# Autodesk Inventor assembly: robotface
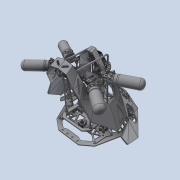
[picture p0: Inventor's stored thumbnail of the model, 180x180]
Saved by Autodesk Inventor 2020 (Build 240168000, 168)
## iProperties
Created: 2021-06-30
Part Number: robotface
Document SubType Name: Assembly
Designer: valer
Author: valer
## Documents named in this file (47)
- C:\Users\Val\Desktop\drummingrobot\design\robotface\robotface.iam
- C:\Users\Val\Desktop\drummingrobot\design\robotface\robotface-final.ipt
- C:\Users\Val\Desktop\drummingrobot\src\parts\external\HingedThreadedStandoffPart2.ipt
- C:\Users\Val\Desktop\drummingrobot\src\parts\external\HingedThreadedStandoffPart1.ipt
- C:\Users\Val\Desktop\drummingrobot\design\robotface\TongueMount.ipt
- C:\Users\Val\Desktop\drummingrobot\design\robotface\HeadMount.ipt
- C:\Users\Val\Desktop\drummingrobot\design\robotface\LinearBearing-1612-0612-0035.ipt
- C:\Users\Val\Desktop\drummingrobot\design\robotface\ClampingHub1301-0016-0012.ipt
- C:\Users\Val\Desktop\drummingrobot\design\robotface\UJoint6D\UJoint6D-Body-4003-1006-1006.ipt
- C:\Users\Val\Desktop\drummingrobot\design\robotface\UJoint6D\UJoint6D-CenterDrive-4003-1006-1006.ipt
- C:\Users\Val\Desktop\drummingrobot\design\robotface\UJoint6D\UJoint6D-Screw.ipt
- C:\Users\Val\Desktop\drummingrobot\design\robotface\SetScrewLiteHub-1308-0016-0006.ipt
- C:\Users\Val\Desktop\drummingrobot\design\robotface\ShaftD6-Short-2101-0006-0020.ipt
- C:\Users\Val\Desktop\drummingrobot\design\robotface\SetScrewHub-1300-0016-1006.ipt
- C:\Users\Val\Desktop\drummingrobot\design\robotface\ShaftD6Female-632Female.ipt
- C:\Users\Val\Desktop\drummingrobot\design\robotface\ShaftD6-2101-0006-0160.ipt
- C:\Users\Val\Desktop\drummingrobot\design\robotface\HeadTongueMount.ipt
- C:\Users\Val\Desktop\drummingrobot\design\robotface\Rod4mm.ipt
- C:\Users\Val\Desktop\drummingrobot\design\robotface\NoseBentBar.ipt
- C:\Users\Val\Desktop\drummingrobot\design\robotface\HeadTopConnector.ipt
- C:\Users\Val\Desktop\drummingrobot\design\robotface\UJointSq-4005-0016-0001\4005-0016-0001 Outer Shell.ipt
- C:\Users\Val\Desktop\drummingrobot\design\robotface\RodEndFixed-2434K495_CORROSION-RESISTANT FULLY THREADED ROD END BOLT.ipt
- C:\Users\Val\Desktop\drummingrobot\design\robotface\StandoffM4-1501-0006-0420.ipt
- C:\Users\Val\Desktop\drummingrobot\design\robotface\StandoffM4-1501-0006-0340.ipt
- C:\Users\Val\Desktop\drummingrobot\src\parts\external\Arducam.ipt
- C:\Users\Val\Desktop\drummingrobot\src\parts\external\ArducamHat.ipt
- C:\Users\Val\Desktop\drummingrobot\design\robotface\HeadEyeMount.ipt
- C:\Users\Val\Desktop\drummingrobot\design\robotface\M3-Standoff-30mm.ipt
- C:\Users\Val\Desktop\drummingrobot\design\robotface\M5-Standoff-32mm.ipt
- C:\Users\Val\Desktop\drummingrobot\src\parts\external\ArducamMirror.ipt
- C:\Users\Val\Desktop\drummingrobot\design\robotface\M1-Standoff-20mm.ipt
- C:\Users\Val\Desktop\drummingrobot\design\robotface\NoseInsideConnector.ipt
- C:\Users\Val\Desktop\drummingrobot\design\robotface\Part2^3mm U-Joint.ipt
- C:\Users\Val\Desktop\drummingrobot\design\robotface\Part1^3mm U-Joint.ipt
- C:\Users\Val\Desktop\drummingrobot\design\robotface\NoseCover.ipt
- C:\Users\Val\Desktop\drummingrobot\design\robotface\NoseCoverSmall.ipt
- C:\Users\Val\Desktop\drummingrobot\design\robotface\IRLed-FY-4006.ipt
- C:\Users\Val\Desktop\drummingrobot\design\robotface\BackEyeMountLeft.ipt
- C:\Users\Val\Desktop\drummingrobot\design\robotface\BackEyeMountRight.ipt
- C:\Users\Val\Desktop\drummingrobot\design\robotface\ShaftClamp6-6058N14.ipt
- C:\Users\Val\Desktop\drummingrobot\design\robotface\MuzzleHeadMount.ipt
- C:\Users\Val\Desktop\drummingrobot\design\robotface\ShaftD6-2100-0006-0200.ipt
- C:\Users\Val\Desktop\drummingrobot\design\robotface\MuzzleHeadConnector.ipt
- C:\Users\Val\Desktop\drummingrobot\src\parts\VacuumTubeHolder.iam
- C:\Users\Val\Desktop\drummingrobot\src\parts\FaceTubeConnector.ipt
- C:\Users\Val\Desktop\drummingrobot\design\robotface\IRLedMount.ipt
- C:\Users\Val\Desktop\drummingrobot\design\robotface\robotface-final-jaw.ipt
## Components (135 placed, 46 different names)
1. robotface-final:1 — Mate:7, Mate:8, Mate:9, Mate:10, Mate:11, Mate:12, Angle:3, Mate:18, Mate:19, Mate:20, Mate:25, Mate:26, Mate:90, Mate:91, Mate:92, Mate:93, Angle:18, Angle:20, Mate:132, Mate:133, Angle:28, Mate:189, Mate:190, Angle:35, Angle:36, Mate:205, Angle:41, Mate:242, Mate:244, Mate:245, Mate:246, Mate:247, Mate:248, Mate:249, Mate:250, Mate:251, Mate:254, Mate:255, Angle:47, Mate:277, Mate:278, Mate:282, Mate:368, Mate:369, Angle:58, Mate:380, Mate:381, Mate:382, Mate:383, Mate:386, Mate:387, Mate:389, Mate:404, Mate:405, Mate:414, Mate:415, Mate:416, Mate:417, Mate:418, Mate:419, Mate:463, Mate:465, Mate:469, Mate:474, Mate:509, Mate:512, Mate:517
2. HingedThreadedStandoffPart2:1 — Mate:1, Mate:2, Flush:1, Angle:4, Mate:284
3. HingedThreadedStandoffPart1:1 — Mate:1, Mate:2, Mate:7, Mate:8
4. HingedThreadedStandoffPart2:2 — Mate:3, Mate:4, Mate:9, Mate:10
5. HingedThreadedStandoffPart1:2 — Mate:3, Mate:4, Flush:1
6. HingedThreadedStandoffPart2:3 — Mate:5, Mate:6, Mate:11, Mate:12, Angle:3, Mate:60, Mate:61
7. HingedThreadedStandoffPart1:3 — Mate:5, Mate:6, Angle:4
8. HingedThreadedStandoffPart2:4 — Mate:18, Mate:19, Mate:20, Mate:21, Mate:22
9. HingedThreadedStandoffPart1:4 — Mate:21, Mate:22, Mate:89
10. HingedThreadedStandoffPart2:5 — Mate:25, Mate:26
11. HingedThreadedStandoffPart1:5 — Mate:85, Mate:86
12. TongueMount:2 — Mate:278, Mate:281, Mate:283, Mate:284, Flush:24
13. HeadMount:1 — Mate:110, Mate:111, Mate:112, Flush:12, Mate:210, Mate:211, Mate:214, Mate:215, Mate:342, Mate:345, Mate:346, Mate:347, Mate:392, Mate:393, Mate:394, Mate:398, Mate:399, Mate:400
14. LinearBearing-1612-0612-0035:1 — Mate:300, Flush:25
15. ClampingHub1301-0016-0012:1 — Mate:115, Mate:282, Mate:300, Flush:25
16. SetScrewLiteHub-1308-0016-0006:1 — Mate:65, Mate:67, Mate:281, Angle:53, Flush:24
17. HingedThreadedStandoffPart2:6 — Mate:60, Mate:61, Mate:283
18. ShaftD6-Short-2101-0006-0020:1 — Mate:65, Mate:67, Angle:51, Mate:297, Flush:22
19. ShaftD6-2101-0006-0160:2 — Mate:87, Angle:16
20. ShaftD6-2101-0006-0160:3
21. SetScrewHub-1300-0016-1006:1
22. SetScrewHub-1300-0016-1006:2
23. ShaftD6Female-632Female:1 — Mate:85, Mate:86
24. ShaftD6Female-632Female:2 — Mate:87, Mate:89, Angle:16
25. HingedThreadedStandoffPart2:9 — Mate:92, Mate:93, Mate:96, Mate:97
26. HingedThreadedStandoffPart2:10 — Mate:90, Mate:91, Mate:94, Mate:95
27. HingedThreadedStandoffPart2:11 — Mate:94, Mate:95, Mate:98, Mate:99
28. HingedThreadedStandoffPart2:12 — Mate:96, Mate:97, Mate:100, Mate:101
29. ShaftD6Female-632Female:3 — Mate:98, Mate:99, Mate:102, Angle:17, Mate:103, Angle:18
30. ShaftD6Female-632Female:4 — Mate:100, Mate:101, Mate:104, Angle:19, Angle:20, Mate:105
31. ShaftD6-2101-0006-0160:4 — Mate:102, Angle:17, Mate:103, Mate:106, Angle:21
32. ShaftD6-2101-0006-0160:5 — Mate:104, Angle:19, Mate:105, Mate:107, Angle:22
33. SetScrewHub-1300-0016-1006:3 — Mate:106, Angle:21, Mate:116
34. SetScrewHub-1300-0016-1006:4 — Mate:107, Angle:22
35. HeadTongueMount:1 — Mate:110, Mate:111, Mate:112, Mate:115, Mate:116, Mate:204, Mate:483
36. Rod4mm:1 — Mate:132
37. Rod4mm:2 — Mate:133
38. SetScrewLiteHub-1308-0016-0006:2 — Mate:151, Flush:5, Mate:153, Angle:26, Mate:242, Mate:370, Mate:371
39. UJoint6D-Body-4003-1006-1006:5 — Angle:28
40. UJoint6D-CenterDrive-4003-1006-1006:3
41. UJoint6D-Screw:11
42. UJoint6D-Body-4003-1006-1006:6 — Mate:152, Angle:25, Mate:153, Angle:26
43. UJoint6D-Screw:12
44. UJoint6D-Screw:13
45. UJoint6D-Screw:14
46. ShaftD6-Short-2101-0006-0020:2 — Mate:151, Flush:5, Mate:152, Angle:25
47. NoseBentBar:1 — Mate:189, Angle:36, Flush:13, Flush:14
48. NoseBentBar:2 — Mate:190, Angle:35, Flush:13
49. HeadTopConnector:1 — Flush:12, Flush:14
50. 4005-0016-0001 Outer Shell:1 — Mate:204, Mate:205
51. RodEndFixed-2434K495_CORROSION-RESISTANT FULLY THREADED ROD END BOLT:1 — Mate:210, Mate:211, Angle:41, Angle:42
52. RodEndFixed-2434K495_CORROSION-RESISTANT FULLY THREADED ROD END BOLT:3 — Mate:214, Mate:215, Angle:42
53. StandoffM4-1501-0006-0420:1 — Mate:244, Mate:245
54. StandoffM4-1501-0006-0420:2 — Mate:246, Mate:247
55. StandoffM4-1501-0006-0340:1 — Mate:248, Mate:249
56. StandoffM4-1501-0006-0340:2 — Mate:250, Mate:251
57. HingedThreadedStandoffPart2:13 — Mate:256, Mate:257
58. HingedThreadedStandoffPart1:6 — Mate:254, Mate:255, Angle:47
59. ShaftD6Female-632Female:5 — Mate:256, Mate:257
60. ArducamHat:1 — Mate:314, Mate:316, Mate:317, Mate:318, Mate:319
61. Arducam:2 — Mate:350, Mate:351, Mate:352, Mate:354, Mate:356, Mate:364, Mate:390, Mate:503, Mate:504, Mate:506, Mate:507
62. HeadEyeMount:1 — Mate:277, Mate:315, Mate:320, Mate:341, Mate:343, Mate:344, Mate:348, Mate:349, Mate:350, Mate:351, Mate:353, Mate:355, Mate:357, Mate:359, Mate:360, Mate:362, Mate:365, Mate:367
63. UJoint6D-Body-4003-1006-1006:12 — Angle:51, Mate:297, Flush:22, Angle:53
64. UJoint6D-Screw:24
65. UJoint6D-Screw:26
66. M3-Standoff-30mm:1 — Mate:314, Mate:315, Mate:316
67. M3-Standoff-30mm:2 — Mate:317, Mate:318
68. M3-Standoff-30mm:3 — Mate:319, Mate:320
69. M5-Standoff-32mm:1 — Mate:341, Mate:342, Mate:343
70. M5-Standoff-32mm:2 — Mate:344, Mate:345
71. M5-Standoff-32mm:3 — Mate:346, Mate:349
72. M5-Standoff-32mm:4 — Mate:347, Mate:348
73. ArducamMirror:1 — Mate:358, Mate:361, Mate:363, Mate:366, Mate:391, Mate:496, Mate:497, Mate:498, Mate:500, Mate:501
74. M1-Standoff-20mm:1 — Mate:352, Mate:353
75. M1-Standoff-20mm:2 — Mate:354, Mate:355, Mate:364
76. M1-Standoff-20mm:3 — Mate:356, Mate:357
77. M1-Standoff-20mm:4 — Mate:358, Mate:359, Mate:360
78. M1-Standoff-20mm:5 — Mate:361, Mate:362, Mate:363, Mate:365
79. M1-Standoff-20mm:6 — Mate:366, Mate:367
80. NoseInsideConnector:1 — Mate:368, Mate:369, Angle:58, Mate:370, Mate:371
81. Part2^3mm U-Joint:1 — Mate:372, Mate:373, Mate:374, Mate:375
82. Part1^3mm U-Joint:1 — Mate:372, Mate:373
83. Part1^3mm U-Joint:2 — Mate:374, Mate:375, Mate:380, Mate:381
84. Part2^3mm U-Joint:2
85. Part1^3mm U-Joint:3
86. Part1^3mm U-Joint:4 — Mate:382, Mate:383
87. NoseCover:1 — Mate:386, Mate:387, Flush:29, Mate:388
88. NoseCoverSmall:1 — Flush:29, Mate:388, Mate:389
89. IRLed-FY-4006:1 — Mate:391, Mate:496, Mate:499, Mate:502, Flush:34
90. IRLed-FY-4006:2 — Mate:390, Flush:34, Mate:505, Mate:508
91. IRLed-FY-4006:3 — Mate:395, Mate:396, Mate:397
92. BackEyeMountRight:1 — Mate:398, Mate:399, Mate:400, Mate:401, Mate:402, Mate:403
93. BackEyeMountLeft:1 — Mate:392, Mate:393, Mate:394, Mate:395, Mate:396, Mate:397
94. IRLed-FY-4006:4 — Mate:401, Mate:402, Mate:403
95. ShaftD6-2100-0006-0200:1 — Mate:432, Mate:436, Mate:482
96. ShaftClamp6-6058N14:1 — Mate:404, Mate:405
97. ShaftD6-2100-0006-0200:2 — Mate:441, Mate:443, Mate:458
98. ShaftClamp6-6058N14:2 — Mate:464
99. ShaftD6-2100-0006-0200:3 — Mate:445, Mate:447, Mate:466
100. ShaftClamp6-6058N14:3
101. ShaftClamp6-6058N14:4 — Mate:414, Mate:415
102. ShaftClamp6-6058N14:5 — Mate:416, Mate:417
103. ShaftD6-2100-0006-0200:4 — Mate:437, Mate:439, Mate:480
104. ShaftClamp6-6058N14:6 — Mate:418, Mate:419
105. ShaftD6-2100-0006-0200:5 — Mate:449, Mate:451, Mate:475
106. ShaftClamp6-6058N14:7 — Mate:476
107. ShaftD6-2100-0006-0200:6 — Mate:453, Mate:455, Mate:470
108. ShaftClamp6-6058N14:8 — Mate:471
109. MuzzleHeadMount:1 — Mate:428, Mate:429, Mate:480, Mate:481, Mate:482, Mate:484, Mate:485, Mate:486, Mate:487, Mate:488, Mate:489, Mate:490, Mate:491, Mate:492, Mate:493, Mate:494, Mate:495
110. MuzzleHeadConnector:1 — Mate:428, Mate:429, Mate:481, Mate:483
111. ShaftClamp6-6058N14:9 — Mate:432, Mate:485
112. ShaftClamp6-6058N14:10 — Mate:436, Mate:486
113. ShaftClamp6-6058N14:12 — Mate:437, Mate:487
114. ShaftClamp6-6058N14:13 — Mate:439, Mate:484
115. ShaftClamp6-6058N14:14 — Mate:441, Mate:492
116. ShaftClamp6-6058N14:15 — Mate:443, Mate:493
117. ShaftClamp6-6058N14:16 — Mate:445, Mate:494
118. ShaftClamp6-6058N14:17 — Mate:447, Mate:488
119. ShaftClamp6-6058N14:18 — Mate:449, Mate:495
120. ShaftClamp6-6058N14:19 — Mate:451, Mate:491
121. ShaftClamp6-6058N14:20 — Mate:453, Mate:490
122. ShaftClamp6-6058N14:21 — Mate:455, Mate:489
123. VacuumTubeHolder:1 [sub-assembly] — Mate:467, Mate:468
124. VacuumTubeHolder:2 [sub-assembly] — Mate:461, Mate:462
125. VacuumTubeHolder:3 [sub-assembly] — Mate:477, Mate:478
126. VacuumTubeHolder:4 [sub-assembly] — Mate:472, Mate:473
127. BackSideConnector:1 — Mate:458, Mate:461, Mate:462, Mate:463, Mate:464
128. BackSideConnector:2 — Mate:465, Mate:466, Mate:467, Mate:468
129. BackSideConnector:3 — Mate:469, Mate:470, Mate:471, Mate:472, Mate:473
130. BackSideConnector:4 — Mate:474, Mate:475, Mate:476, Mate:477, Mate:478
131. IRLedMount:1 — Mate:500, Mate:501, Mate:502
132. IRLedMount:2 — Mate:497, Mate:498, Mate:499
133. IRLedMount:3 — Mate:506, Mate:507, Mate:508
134. IRLedMount:4 — Mate:503, Mate:504, Mate:505
135. robotface-final-jaw:1 — Mate:510, Mate:515, Mate:517
## Relationships (309: Mate 268, Angle 27, Flush 14)
- Mate:1: HingedThreadedStandoffPart2:1 ↔ HingedThreadedStandoffPart1:1
- Mate:2: HingedThreadedStandoffPart2:1 ↔ HingedThreadedStandoffPart1:1
- Mate:3: HingedThreadedStandoffPart2:2 ↔ HingedThreadedStandoffPart1:2
- Mate:4: HingedThreadedStandoffPart2:2 ↔ HingedThreadedStandoffPart1:2
- Mate:5: HingedThreadedStandoffPart2:3 ↔ HingedThreadedStandoffPart1:3
- Mate:6: HingedThreadedStandoffPart2:3 ↔ HingedThreadedStandoffPart1:3
- Mate:7: robotface-final:1 ↔ HingedThreadedStandoffPart1:1
- Mate:8: robotface-final:1 ↔ HingedThreadedStandoffPart1:1
- Mate:9: robotface-final:1 ↔ HingedThreadedStandoffPart2:2
- Mate:10: robotface-final:1 ↔ HingedThreadedStandoffPart2:2
- Mate:11: robotface-final:1 ↔ HingedThreadedStandoffPart2:3
- Mate:12: robotface-final:1 ↔ HingedThreadedStandoffPart2:3
- Angle:3 (0 deg): robotface-final:1 ↔ HingedThreadedStandoffPart2:3
- Mate:18: robotface-final:1 ↔ HingedThreadedStandoffPart2:4
- Mate:19: robotface-final:1 ↔ HingedThreadedStandoffPart2:4
- Mate:20: robotface-final:1 ↔ HingedThreadedStandoffPart2:4
- Mate:21: HingedThreadedStandoffPart2:4 ↔ HingedThreadedStandoffPart1:4
- Mate:22: HingedThreadedStandoffPart2:4 ↔ HingedThreadedStandoffPart1:4
- [Mate]: HingedThreadedStandoffPart2:5 ↔ HingedThreadedStandoffPart1:5
- [Mate]: HingedThreadedStandoffPart2:5 ↔ HingedThreadedStandoffPart1:5
- Mate:25: robotface-final:1 ↔ HingedThreadedStandoffPart2:5
- Mate:26: robotface-final:1 ↔ HingedThreadedStandoffPart2:5
- Flush:1: HingedThreadedStandoffPart2:1 ↔ HingedThreadedStandoffPart1:2
- Angle:4 (0 deg): HingedThreadedStandoffPart2:1 ↔ HingedThreadedStandoffPart1:3
- Mate:60: HingedThreadedStandoffPart2:3 ↔ HingedThreadedStandoffPart2:6
- Mate:61: HingedThreadedStandoffPart2:3 ↔ HingedThreadedStandoffPart2:6
- Mate:65: SetScrewLiteHub-1308-0016-0006:1 ↔ ShaftD6-Short-2101-0006-0020:1
- Mate:67 (-7 mm): SetScrewLiteHub-1308-0016-0006:1 ↔ ShaftD6-Short-2101-0006-0020:1
- [Mate]: HingedThreadedStandoffPart1:4 ↔ ShaftD6-2101-0006-0160:2
- [Angle] (0 deg): HeadMount:1 ↔ ShaftD6-2101-0006-0160:2
- [Mate]: HingedThreadedStandoffPart1:5 ↔ ShaftD6-2101-0006-0160:3
- [Angle] (0 deg): HeadMount:1 ↔ ShaftD6-2101-0006-0160:3
- [Mate]: ShaftD6-2101-0006-0160:2 ↔ SetScrewHub-1300-0016-1006:1
- [Mate]: ShaftD6-2101-0006-0160:3 ↔ SetScrewHub-1300-0016-1006:2
- [Angle] (0 deg): ShaftD6-2101-0006-0160:2 ↔ SetScrewHub-1300-0016-1006:1
- [Angle] (0 deg): ShaftD6-2101-0006-0160:3 ↔ SetScrewHub-1300-0016-1006:2
- [Angle] (0 deg): robotface-final:1 ↔ ShaftD6-2101-0006-0160:2
- [Angle] (0 deg): robotface-final:1 ↔ ShaftD6-2101-0006-0160:3
- [Mate]: ShaftD6-2101-0006-0160:3 ↔ ShaftD6Female-632Female:1
- [Angle] (0 deg): ShaftD6-2101-0006-0160:3 ↔ ShaftD6Female-632Female:1
- [Mate]: ShaftD6-2101-0006-0160:3 ↔ ShaftD6Female-632Female:1
- Mate:85: HingedThreadedStandoffPart1:5 ↔ ShaftD6Female-632Female:1
- Mate:86: HingedThreadedStandoffPart1:5 ↔ ShaftD6Female-632Female:1
- Mate:87: ShaftD6-2101-0006-0160:2 ↔ ShaftD6Female-632Female:2
- Mate:89: HingedThreadedStandoffPart1:4 ↔ ShaftD6Female-632Female:2
- Angle:16 (0 deg): ShaftD6-2101-0006-0160:2 ↔ ShaftD6Female-632Female:2
- Mate:90: robotface-final:1 ↔ HingedThreadedStandoffPart2:10
- Mate:91: robotface-final:1 ↔ HingedThreadedStandoffPart2:10
- Mate:92: robotface-final:1 ↔ HingedThreadedStandoffPart2:9
- Mate:93: robotface-final:1 ↔ HingedThreadedStandoffPart2:9
- Mate:94: HingedThreadedStandoffPart2:10 ↔ HingedThreadedStandoffPart2:11
- Mate:95: HingedThreadedStandoffPart2:10 ↔ HingedThreadedStandoffPart2:11
- Mate:96: HingedThreadedStandoffPart2:9 ↔ HingedThreadedStandoffPart2:12
- Mate:97: HingedThreadedStandoffPart2:9 ↔ HingedThreadedStandoffPart2:12
- Mate:98: HingedThreadedStandoffPart2:11 ↔ ShaftD6Female-632Female:3
- Mate:99: HingedThreadedStandoffPart2:11 ↔ ShaftD6Female-632Female:3
- Mate:100: HingedThreadedStandoffPart2:12 ↔ ShaftD6Female-632Female:4
- Mate:101: HingedThreadedStandoffPart2:12 ↔ ShaftD6Female-632Female:4
- Mate:102: ShaftD6Female-632Female:3 ↔ ShaftD6-2101-0006-0160:4
- Angle:17 (0 deg): ShaftD6Female-632Female:3 ↔ ShaftD6-2101-0006-0160:4
- Mate:103: ShaftD6Female-632Female:3 ↔ ShaftD6-2101-0006-0160:4
- Angle:18 (180 deg): robotface-final:1 ↔ ShaftD6Female-632Female:3
- Mate:104: ShaftD6Female-632Female:4 ↔ ShaftD6-2101-0006-0160:5
- Angle:19 (0 deg): ShaftD6Female-632Female:4 ↔ ShaftD6-2101-0006-0160:5
- Angle:20 (180 deg): robotface-final:1 ↔ ShaftD6Female-632Female:4
- Mate:105: ShaftD6Female-632Female:4 ↔ ShaftD6-2101-0006-0160:5
- Mate:106: ShaftD6-2101-0006-0160:4 ↔ SetScrewHub-1300-0016-1006:3
- Angle:21 (180 deg): ShaftD6-2101-0006-0160:4 ↔ SetScrewHub-1300-0016-1006:3
- Mate:107: ShaftD6-2101-0006-0160:5 ↔ SetScrewHub-1300-0016-1006:4
- Angle:22 (180 deg): ShaftD6-2101-0006-0160:5 ↔ SetScrewHub-1300-0016-1006:4
- Mate:110: HeadMount:1 ↔ HeadTongueMount:1
- Mate:111: HeadMount:1 ↔ HeadTongueMount:1
- Mate:112: HeadMount:1 ↔ HeadTongueMount:1
- Mate:115: ClampingHub1301-0016-0012:1 ↔ HeadTongueMount:1
- Mate:116: SetScrewHub-1300-0016-1006:3 ↔ HeadTongueMount:1
- Mate:132: robotface-final:1 ↔ Rod4mm:1
- Mate:133: robotface-final:1 ↔ Rod4mm:2
- [Mate]: UJoint6D-CenterDrive-4003-1006-1006:3 ↔ UJoint6D-Body-4003-1006-1006:6
- [Mate]: UJoint6D-CenterDrive-4003-1006-1006:3 ↔ UJoint6D-Body-4003-1006-1006:6
- [Mate]: UJoint6D-Body-4003-1006-1006:5 ↔ UJoint6D-CenterDrive-4003-1006-1006:3
- [Mate]: UJoint6D-Body-4003-1006-1006:5 ↔ UJoint6D-CenterDrive-4003-1006-1006:3
- [Mate]: UJoint6D-Body-4003-1006-1006:5 ↔ UJoint6D-Screw:11
- [Mate]: UJoint6D-Body-4003-1006-1006:5 ↔ UJoint6D-Screw:11
- [Mate]: UJoint6D-Body-4003-1006-1006:5 ↔ UJoint6D-Screw:13
- [Mate]: UJoint6D-Body-4003-1006-1006:5 ↔ UJoint6D-Screw:13
- [Mate]: UJoint6D-Body-4003-1006-1006:6 ↔ UJoint6D-Screw:12
- [Mate]: UJoint6D-Body-4003-1006-1006:6 ↔ UJoint6D-Screw:12
- [Mate]: UJoint6D-Body-4003-1006-1006:6 ↔ UJoint6D-Screw:14
- [Mate]: UJoint6D-Body-4003-1006-1006:6 ↔ UJoint6D-Screw:14
- Mate:151: SetScrewLiteHub-1308-0016-0006:2 ↔ ShaftD6-Short-2101-0006-0020:2
- Flush:5: SetScrewLiteHub-1308-0016-0006:2 ↔ ShaftD6-Short-2101-0006-0020:2
- Mate:152: UJoint6D-Body-4003-1006-1006:6 ↔ ShaftD6-Short-2101-0006-0020:2
- Angle:25 (180 deg): UJoint6D-Body-4003-1006-1006:6 ↔ ShaftD6-Short-2101-0006-0020:2
- Mate:153: SetScrewLiteHub-1308-0016-0006:2 ↔ UJoint6D-Body-4003-1006-1006:6
- Angle:26 (0 deg): SetScrewLiteHub-1308-0016-0006:2 ↔ UJoint6D-Body-4003-1006-1006:6
- Angle:28 (0 deg): robotface-final:1 ↔ UJoint6D-Body-4003-1006-1006:5
- Mate:189: robotface-final:1 ↔ NoseBentBar:1
- Mate:190: robotface-final:1 ↔ NoseBentBar:2
- Flush:12: HeadMount:1 ↔ HeadTopConnector:1
- Angle:35 (0 deg): robotface-final:1 ↔ NoseBentBar:2
- Angle:36 (0 deg): robotface-final:1 ↔ NoseBentBar:1
- Flush:13: NoseBentBar:1 ↔ NoseBentBar:2
- Flush:14: NoseBentBar:1 ↔ HeadTopConnector:1
- Mate:204: HeadTongueMount:1 ↔ 4005-0016-0001 Outer Shell:1
- Mate:205: robotface-final:1 ↔ 4005-0016-0001 Outer Shell:1
- Mate:210: HeadMount:1 ↔ RodEndFixed-2434K495_CORROSION-RESISTANT FULLY THREADED ROD END BOLT:1
- Mate:211 (-17.78 mm): HeadMount:1 ↔ RodEndFixed-2434K495_CORROSION-RESISTANT FULLY THREADED ROD END BOLT:1
- Angle:41 (0 deg): robotface-final:1 ↔ RodEndFixed-2434K495_CORROSION-RESISTANT FULLY THREADED ROD END BOLT:1
- Mate:214: HeadMount:1 ↔ RodEndFixed-2434K495_CORROSION-RESISTANT FULLY THREADED ROD END BOLT:3
- Mate:215 (-17.78 mm): HeadMount:1 ↔ RodEndFixed-2434K495_CORROSION-RESISTANT FULLY THREADED ROD END BOLT:3
- Angle:42 (0 deg): RodEndFixed-2434K495_CORROSION-RESISTANT FULLY THREADED ROD END BOLT:1 ↔ RodEndFixed-2434K495_CORROSION-RESISTANT FULLY THREADED ROD END BOLT:3
- Mate:242: robotface-final:1 ↔ SetScrewLiteHub-1308-0016-0006:2
- Mate:244: robotface-final:1 ↔ StandoffM4-1501-0006-0420:1
- Mate:245: robotface-final:1 ↔ StandoffM4-1501-0006-0420:1
- Mate:246: robotface-final:1 ↔ StandoffM4-1501-0006-0420:2
- Mate:247: robotface-final:1 ↔ StandoffM4-1501-0006-0420:2
- Mate:248: robotface-final:1 ↔ StandoffM4-1501-0006-0340:1
- Mate:249: robotface-final:1 ↔ StandoffM4-1501-0006-0340:1
- Mate:250: robotface-final:1 ↔ StandoffM4-1501-0006-0340:2
- Mate:251: robotface-final:1 ↔ StandoffM4-1501-0006-0340:2
- [Mate]: HingedThreadedStandoffPart2:13 ↔ HingedThreadedStandoffPart1:6
- [Mate]: HingedThreadedStandoffPart2:13 ↔ HingedThreadedStandoffPart1:6
- Mate:254: robotface-final:1 ↔ HingedThreadedStandoffPart1:6
- Mate:255: robotface-final:1 ↔ HingedThreadedStandoffPart1:6
- Angle:47 (0 deg): robotface-final:1 ↔ HingedThreadedStandoffPart1:6
- Mate:256: HingedThreadedStandoffPart2:13 ↔ ShaftD6Female-632Female:5
- Mate:257: HingedThreadedStandoffPart2:13 ↔ ShaftD6Female-632Female:5
- Mate:277: robotface-final:1 ↔ HeadEyeMount:1
- Mate:278: robotface-final:1 ↔ TongueMount:2
- Mate:281: TongueMount:2 ↔ SetScrewLiteHub-1308-0016-0006:1
- Mate:282: robotface-final:1 ↔ ClampingHub1301-0016-0012:1
- Mate:283: TongueMount:2 ↔ HingedThreadedStandoffPart2:6
- Mate:284: HingedThreadedStandoffPart2:1 ↔ TongueMount:2
- [Mate]: UJoint6D-Body-4003-1006-1006:12 ↔ UJoint6D-Screw:24
- [Mate]: UJoint6D-Body-4003-1006-1006:12 ↔ UJoint6D-Screw:24
- [Mate]: UJoint6D-Body-4003-1006-1006:12 ↔ UJoint6D-Screw:26
- [Mate]: UJoint6D-Body-4003-1006-1006:12 ↔ UJoint6D-Screw:26
- Angle:51 (0 deg): ShaftD6-Short-2101-0006-0020:1 ↔ UJoint6D-Body-4003-1006-1006:12
- Mate:297: ShaftD6-Short-2101-0006-0020:1 ↔ UJoint6D-Body-4003-1006-1006:12
- Flush:22: ShaftD6-Short-2101-0006-0020:1 ↔ UJoint6D-Body-4003-1006-1006:12
- Angle:53 (0 deg): SetScrewLiteHub-1308-0016-0006:1 ↔ UJoint6D-Body-4003-1006-1006:12
- Mate:300: LinearBearing-1612-0612-0035:1 ↔ ClampingHub1301-0016-0012:1
- Flush:24: TongueMount:2 ↔ SetScrewLiteHub-1308-0016-0006:1
- Flush:25 (6 mm): LinearBearing-1612-0612-0035:1 ↔ ClampingHub1301-0016-0012:1
- Mate:314: ArducamHat:1 ↔ M3-Standoff-30mm:1
- Mate:315: HeadEyeMount:1 ↔ M3-Standoff-30mm:1
- Mate:316: ArducamHat:1 ↔ M3-Standoff-30mm:1
- Mate:317: ArducamHat:1 ↔ M3-Standoff-30mm:2
- Mate:318: ArducamHat:1 ↔ M3-Standoff-30mm:2
- Mate:319: ArducamHat:1 ↔ M3-Standoff-30mm:3
- Mate:320: HeadEyeMount:1 ↔ M3-Standoff-30mm:3
- Mate:341: HeadEyeMount:1 ↔ M5-Standoff-32mm:1
- Mate:342: HeadMount:1 ↔ M5-Standoff-32mm:1
- Mate:343: HeadEyeMount:1 ↔ M5-Standoff-32mm:1
- Mate:344: HeadEyeMount:1 ↔ M5-Standoff-32mm:2
- Mate:345: HeadMount:1 ↔ M5-Standoff-32mm:2
- Mate:346: HeadMount:1 ↔ M5-Standoff-32mm:3
- Mate:347: HeadMount:1 ↔ M5-Standoff-32mm:4
- Mate:348: HeadEyeMount:1 ↔ M5-Standoff-32mm:4
- Mate:349: HeadEyeMount:1 ↔ M5-Standoff-32mm:3
- Mate:350: Arducam:2 ↔ HeadEyeMount:1
- Mate:351: Arducam:2 ↔ HeadEyeMount:1
- Mate:352: Arducam:2 ↔ M1-Standoff-20mm:1
- Mate:353: HeadEyeMount:1 ↔ M1-Standoff-20mm:1
- Mate:354: Arducam:2 ↔ M1-Standoff-20mm:2
- Mate:355: HeadEyeMount:1 ↔ M1-Standoff-20mm:2
- Mate:356: Arducam:2 ↔ M1-Standoff-20mm:3
- Mate:357: HeadEyeMount:1 ↔ M1-Standoff-20mm:3
- Mate:358: ArducamMirror:1 ↔ M1-Standoff-20mm:4
- Mate:359: HeadEyeMount:1 ↔ M1-Standoff-20mm:4
- Mate:360: HeadEyeMount:1 ↔ M1-Standoff-20mm:4
- Mate:361: ArducamMirror:1 ↔ M1-Standoff-20mm:5
- Mate:362: HeadEyeMount:1 ↔ M1-Standoff-20mm:5
- Mate:363: ArducamMirror:1 ↔ M1-Standoff-20mm:5
- Mate:364: Arducam:2 ↔ M1-Standoff-20mm:2
- Mate:365: HeadEyeMount:1 ↔ M1-Standoff-20mm:5
- Mate:366: ArducamMirror:1 ↔ M1-Standoff-20mm:6
- Mate:367: HeadEyeMount:1 ↔ M1-Standoff-20mm:6
- Mate:368: robotface-final:1 ↔ NoseInsideConnector:1
- Mate:369: robotface-final:1 ↔ NoseInsideConnector:1
- Angle:58 (0 deg): robotface-final:1 ↔ NoseInsideConnector:1
- Mate:370: SetScrewLiteHub-1308-0016-0006:2 ↔ NoseInsideConnector:1
- Mate:371: SetScrewLiteHub-1308-0016-0006:2 ↔ NoseInsideConnector:1
- Mate:372: Part2^3mm U-Joint:1 ↔ Part1^3mm U-Joint:1
- Mate:373 (0.15 mm): Part2^3mm U-Joint:1 ↔ Part1^3mm U-Joint:1
- Mate:374: Part2^3mm U-Joint:1 ↔ Part1^3mm U-Joint:2
- Mate:375 (0.15 mm): Part2^3mm U-Joint:1 ↔ Part1^3mm U-Joint:2
- [Mate]: Part2^3mm U-Joint:2 ↔ Part1^3mm U-Joint:3
- [Mate] (0.15 mm): Part2^3mm U-Joint:2 ↔ Part1^3mm U-Joint:3
- [Mate]: Part2^3mm U-Joint:2 ↔ Part1^3mm U-Joint:4
- [Mate] (0.15 mm): Part2^3mm U-Joint:2 ↔ Part1^3mm U-Joint:4
- Mate:380: robotface-final:1 ↔ Part1^3mm U-Joint:2
- Mate:381: robotface-final:1 ↔ Part1^3mm U-Joint:2
- Mate:382: robotface-final:1 ↔ Part1^3mm U-Joint:4
- Mate:383: robotface-final:1 ↔ Part1^3mm U-Joint:4
- Mate:386: robotface-final:1 ↔ NoseCover:1
- Mate:387: robotface-final:1 ↔ NoseCover:1
- Flush:29: NoseCover:1 ↔ NoseCoverSmall:1
- Mate:388 (10 mm): NoseCover:1 ↔ NoseCoverSmall:1
- Mate:389: robotface-final:1 ↔ NoseCoverSmall:1
- Mate:390: Arducam:2 ↔ IRLed-FY-4006:2
- Mate:391: ArducamMirror:1 ↔ IRLed-FY-4006:1
- Mate:392: HeadMount:1 ↔ BackEyeMountLeft:1
- Mate:393: HeadMount:1 ↔ BackEyeMountLeft:1
- Mate:394: HeadMount:1 ↔ BackEyeMountLeft:1
- Mate:395: IRLed-FY-4006:3 ↔ BackEyeMountLeft:1
- Mate:396: IRLed-FY-4006:3 ↔ BackEyeMountLeft:1
- Mate:397: IRLed-FY-4006:3 ↔ BackEyeMountLeft:1
- Mate:398: HeadMount:1 ↔ BackEyeMountRight:1
- Mate:399: HeadMount:1 ↔ BackEyeMountRight:1
- Mate:400: HeadMount:1 ↔ BackEyeMountRight:1
- Mate:401: BackEyeMountRight:1 ↔ IRLed-FY-4006:4
- Mate:402: BackEyeMountRight:1 ↔ IRLed-FY-4006:4
- Mate:403: BackEyeMountRight:1 ↔ IRLed-FY-4006:4
- Mate:404: robotface-final:1 ↔ ShaftClamp6-6058N14:1
- Mate:405: robotface-final:1 ↔ ShaftClamp6-6058N14:1
- [Mate]: robotface-final:1 ↔ ShaftD6-2100-0006-0200:1
- [Mate]: robotface-final:1 ↔ ShaftD6-2100-0006-0200:1
- [Mate]: robotface-final:1 ↔ ShaftD6-2100-0006-0200:2
- [Mate]: ShaftD6-2100-0006-0200:2 ↔ ShaftClamp6-6058N14:2
- [Flush]: robotface-final:1 ↔ ShaftD6-2100-0006-0200:2
- [Mate]: ShaftD6-2100-0006-0200:3 ↔ ShaftClamp6-6058N14:3
- [Mate]: robotface-final:1 ↔ ShaftD6-2100-0006-0200:3
- [Flush]: robotface-final:1 ↔ ShaftD6-2100-0006-0200:3
- Mate:414: robotface-final:1 ↔ ShaftClamp6-6058N14:4
- Mate:415: robotface-final:1 ↔ ShaftClamp6-6058N14:4
- Mate:416: robotface-final:1 ↔ ShaftClamp6-6058N14:5
- Mate:417: robotface-final:1 ↔ ShaftClamp6-6058N14:5
- Mate:418: robotface-final:1 ↔ ShaftClamp6-6058N14:6
- Mate:419: robotface-final:1 ↔ ShaftClamp6-6058N14:6
- [Mate]: ShaftD6-2100-0006-0200:4 ↔ ShaftClamp6-6058N14:6
- [Mate]: robotface-final:1 ↔ ShaftD6-2100-0006-0200:4
- [Mate]: ShaftD6-2100-0006-0200:5 ↔ ShaftClamp6-6058N14:7
- [Mate]: robotface-final:1 ↔ ShaftD6-2100-0006-0200:5
- [Flush]: robotface-final:1 ↔ ShaftD6-2100-0006-0200:5
- [Mate]: ShaftD6-2100-0006-0200:6 ↔ ShaftClamp6-6058N14:8
- [Mate]: robotface-final:1 ↔ ShaftD6-2100-0006-0200:6
- [Flush]: robotface-final:1 ↔ ShaftD6-2100-0006-0200:6
- Mate:428: MuzzleHeadMount:1 ↔ MuzzleHeadConnector:1
- Mate:429: MuzzleHeadMount:1 ↔ MuzzleHeadConnector:1
- Mate:432: ShaftD6-2100-0006-0200:1 ↔ ShaftClamp6-6058N14:9
- Mate:436: ShaftD6-2100-0006-0200:1 ↔ ShaftClamp6-6058N14:10
- Mate:437: ShaftD6-2100-0006-0200:4 ↔ ShaftClamp6-6058N14:12
- Mate:439: ShaftD6-2100-0006-0200:4 ↔ ShaftClamp6-6058N14:13
- Mate:441: ShaftD6-2100-0006-0200:2 ↔ ShaftClamp6-6058N14:14
- Mate:443: ShaftD6-2100-0006-0200:2 ↔ ShaftClamp6-6058N14:15
- Mate:445: ShaftD6-2100-0006-0200:3 ↔ ShaftClamp6-6058N14:16
- Mate:447: ShaftD6-2100-0006-0200:3 ↔ ShaftClamp6-6058N14:17
- Mate:449: ShaftD6-2100-0006-0200:5 ↔ ShaftClamp6-6058N14:18
- Mate:451: ShaftD6-2100-0006-0200:5 ↔ ShaftClamp6-6058N14:19
- Mate:453: ShaftD6-2100-0006-0200:6 ↔ ShaftClamp6-6058N14:20
- Mate:455: ShaftD6-2100-0006-0200:6 ↔ ShaftClamp6-6058N14:21
- Mate:458: ShaftD6-2100-0006-0200:2 ↔ BackSideConnector:1
- Mate:461: VacuumTubeHolder:2 ↔ BackSideConnector:1
- Mate:462: VacuumTubeHolder:2 ↔ BackSideConnector:1
- Mate:463: robotface-final:1 ↔ BackSideConnector:1
- Mate:464: ShaftClamp6-6058N14:2 ↔ BackSideConnector:1
- Mate:465: robotface-final:1 ↔ BackSideConnector:2
- Mate:466: ShaftD6-2100-0006-0200:3 ↔ BackSideConnector:2
- Mate:467: VacuumTubeHolder:1 ↔ BackSideConnector:2
- Mate:468: VacuumTubeHolder:1 ↔ BackSideConnector:2
- Mate:469: robotface-final:1 ↔ BackSideConnector:3
- Mate:470: ShaftD6-2100-0006-0200:6 ↔ BackSideConnector:3
- Mate:471: ShaftClamp6-6058N14:8 ↔ BackSideConnector:3
- Mate:472: VacuumTubeHolder:4 ↔ BackSideConnector:3
- Mate:473: VacuumTubeHolder:4 ↔ BackSideConnector:3
- Mate:474: robotface-final:1 ↔ BackSideConnector:4
- Mate:475: ShaftD6-2100-0006-0200:5 ↔ BackSideConnector:4
- Mate:476: ShaftClamp6-6058N14:7 ↔ BackSideConnector:4
- Mate:477: VacuumTubeHolder:3 ↔ BackSideConnector:4
- Mate:478: VacuumTubeHolder:3 ↔ BackSideConnector:4
- Mate:480: ShaftD6-2100-0006-0200:4 ↔ MuzzleHeadMount:1
- Mate:481: MuzzleHeadMount:1 ↔ MuzzleHeadConnector:1
- Mate:482: ShaftD6-2100-0006-0200:1 ↔ MuzzleHeadMount:1
- Mate:483: HeadTongueMount:1 ↔ MuzzleHeadConnector:1
- Mate:484: MuzzleHeadMount:1 ↔ ShaftClamp6-6058N14:13
- Mate:485: MuzzleHeadMount:1 ↔ ShaftClamp6-6058N14:9
- Mate:486: MuzzleHeadMount:1 ↔ ShaftClamp6-6058N14:10
- Mate:487: MuzzleHeadMount:1 ↔ ShaftClamp6-6058N14:12
- Mate:488: MuzzleHeadMount:1 ↔ ShaftClamp6-6058N14:17
- Mate:489: MuzzleHeadMount:1 ↔ ShaftClamp6-6058N14:21
- Mate:490: MuzzleHeadMount:1 ↔ ShaftClamp6-6058N14:20
- Mate:491: MuzzleHeadMount:1 ↔ ShaftClamp6-6058N14:19
- Mate:492: MuzzleHeadMount:1 ↔ ShaftClamp6-6058N14:14
- Mate:493: MuzzleHeadMount:1 ↔ ShaftClamp6-6058N14:15
- Mate:494: MuzzleHeadMount:1 ↔ ShaftClamp6-6058N14:16
- Mate:495: MuzzleHeadMount:1 ↔ ShaftClamp6-6058N14:18
- Mate:496 (7 mm): ArducamMirror:1 ↔ IRLed-FY-4006:1
- Mate:497: ArducamMirror:1 ↔ IRLedMount:2
- Mate:498: ArducamMirror:1 ↔ IRLedMount:2
- Mate:499: IRLed-FY-4006:1 ↔ IRLedMount:2
- Mate:500: ArducamMirror:1 ↔ IRLedMount:1
- Mate:501: ArducamMirror:1 ↔ IRLedMount:1
- Mate:502: IRLed-FY-4006:1 ↔ IRLedMount:1
- Mate:503: Arducam:2 ↔ IRLedMount:4
- Mate:504: Arducam:2 ↔ IRLedMount:4
- Flush:34: IRLed-FY-4006:1 ↔ IRLed-FY-4006:2
- Mate:505: IRLed-FY-4006:2 ↔ IRLedMount:4
- Mate:506: Arducam:2 ↔ IRLedMount:3
- Mate:507: Arducam:2 ↔ IRLedMount:3
- Mate:508: IRLed-FY-4006:2 ↔ IRLedMount:3
- Mate:509: robotface-final:1
- Mate:510: robotface-final-jaw:1
- Mate:511
- Mate:512: robotface-final:1
- Mate:514
- Mate:515: robotface-final-jaw:1
- Mate:516
- Mate:517: robotface-final:1 ↔ robotface-final-jaw:1
## Named parameters: d60_d58 = 0 mm, d61_d59 = 0 mm, d275_d245_d146 = 0 mm, d276_d246_d147 = 0 mm, d277_d247_d148 = 0 mm, d278_d248_d149 = 0 mm, d279_d249_d150 = 0 mm, d280_d250_d151 = 0 mm, d281_d251_d152 = 0 mm, d282_d252_d153 = 0 mm, d283_d253_d154 = 0 mm, d284_d254_d155 = 0 mm, d285_d255_d156 = 0 mm, d286_d256_d157 = 0 mm, d466_d58 = 0 mm, d467_d59 = 0 mm, d520_d253_d154 = 0 mm, d521_d254_d155 = 0 mm, d522_d255_d156 = 0 mm, d523_d256_d157 = 0 mm, d629_d625 = 0 mm, d630_d626 = 0.15 mm, d631_d627 = 0 mm, d632_d628 = 0.15 mm, d678_d675 = 0 mm, d692_d678_d675 = 0 mm, d696_d692_d678_d675 = 0 mm
